# Autodesk Inventor assembly: Hook Assemly Concept
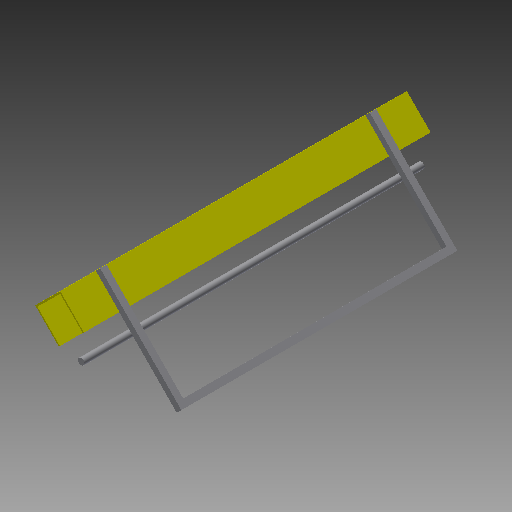
[picture p0: Inventor's stored thumbnail of the model, 512x512]
Saved by Autodesk Inventor 2018 (Build 220112000, 112)
## iProperties
Created: 2018-01-29
Part Number: Hook Assemly Concept
Document SubType Name: Assembly
Designer: Apple
Author: Apple
## Documents named in this file (4)
- C:\Users\Apple\Documents\Inventor\2018 PowerUp\Hook\Hook Assemly Concept.iam
- C:\Users\Apple\Documents\Inventor\2018 PowerUp\2018 Concept Hook.ipt
- C:\Users\Apple\Documents\Inventor\2018 PowerUp\Hook\Hook Concept Cross Bar.ipt
- C:\Users\Apple\Documents\Inventor\2018 PowerUp\Hook\Drop Loop.ipt
## Components (3 placed, 3 different names)
1. 2018 Concept Hook:1 — Flush:1
2. Hook Concept Cross Bar:1 — Tangent:1
3. Drop Loop:1 — Flush:1, Tangent:1
## Relationships (2: Flush 1, Tangent 1)
- Flush:1: 2018 Concept Hook:1 ↔ Drop Loop:1
- Tangent:1: Hook Concept Cross Bar:1 ↔ Drop Loop:1
